# Autodesk Inventor assembly: MG_996R
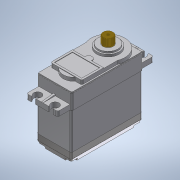
[picture p0: Inventor's stored thumbnail of the model, 180x180]
Saved by Autodesk Inventor 2020 (Build 240168000, 168)
## iProperties
Created: 2016-09-26
Part Number: MG_996R
Document SubType Name: Assembly
Designer: Julian
Author: Julian
## Documents named in this file (5)
- C:\Users\blep\Desktop\ScanBot\3d-model\MG996R servo\MG_996R.iam
- C:\Users\blep\Desktop\ScanBot\3d-model\MG996R servo\Base.ipt
- C:\Users\blep\Desktop\ScanBot\3d-model\MG996R servo\Medio.ipt
- C:\Users\blep\Desktop\ScanBot\3d-model\MG996R servo\Top.ipt
- C:\Users\blep\Desktop\ScanBot\3d-model\MG996R servo\Eje.ipt
## Components (4 placed, 4 different names)
1. Top:1 — Rígido:2, De rotación:1
2. Medio:1 — Rígido:1, Rígido:2
3. Base:1 — Rígido:1
4. Eje:1 — De rotación:1
## Relationships (3: WeldJoint 2, RevoluteJoint 1)
- Rígido:1 [WeldJoint]: Medio:1 ↔ Base:1
- Rígido:2 [WeldJoint]: Top:1 ↔ Medio:1
- De rotación:1 [RevoluteJoint]: Top:1 ↔ Eje:1
